# Autodesk Inventor assembly: Lotus_assembly
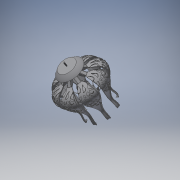
[picture p0: Inventor's stored thumbnail of the model, 180x180]
Saved by Autodesk Inventor 2019 (Build 230136000, 136)
## iProperties
Created: 2019-11-12
Part Number: Lotus_assembly
Document SubType Name: Assembly
Designer: Jorian Brusind
Author: Jorian Brusind
## Documents named in this file (9)
- C:\Users\Jorian Brusind\Documents\GitHub\PersonalProjects\Inventor Projects\Johan\Inventor Files\Lotus_assembly.iam
- C:\Users\Jorian Brusind\Documents\GitHub\PersonalProjects\Inventor Projects\Johan\Inventor Files\Lotus_Petal.ipt
- C:\Users\Jorian Brusind\Documents\GitHub\PersonalProjects\Inventor Projects\Johan\Inventor Files\Ring.ipt
- C:\Users\Jorian Brusind\Documents\GitHub\PersonalProjects\Inventor Projects\Johan\Inventor Files\Leaf.ipt
- C:\Users\Jorian Brusind\Documents\GitHub\PersonalProjects\Inventor Projects\Johan\Inventor Files\inner_ring.ipt
- C:\Users\Jorian Brusind\Documents\GitHub\PersonalProjects\Inventor Projects\Johan\Inventor Files\Innter_petal.ipt
- C:\Users\Jorian Brusind\Documents\GitHub\PersonalProjects\Inventor Projects\Johan\Inventor Files\Threaded_Rod.ipt
- C:\Users\Jorian Brusind\Documents\GitHub\PersonalProjects\Inventor Projects\Johan\Inventor Files\Hex_Center.ipt
- C:\Users\Jorian Brusind\Documents\GitHub\PersonalProjects\Inventor Projects\Johan\Inventor Files\Connector_Rd.ipt
## Components (25 placed, 8 different names)
1. Lotus_Petal:1 — Mate:6, Flush:8, Mate:29
2. Lotus_Petal:2 — Mate:2, Flush:6, Mate:33
3. Lotus_Petal:4 — Mate:4, Flush:1, Mate:27
4. Lotus_Petal:5 — Mate:1, Flush:4, Mate:37
5. Lotus_Petal:6 — Mate:3, Flush:5, Mate:35
6. Lotus_Petal:7 — Mate:5, Flush:7, Mate:31
7. Ring:1 — Mate:1, Mate:2, Mate:3, Mate:4, Mate:5, Mate:6, Mate:7, Mate:8, Flush:1, Flush:2, Flush:3, Flush:4, Flush:5, Flush:6, Flush:7, Flush:8, Mate:9, Mate:10, Mate:11, Mate:12, Mate:19
8. Lotus_Petal:8 — Mate:7, Flush:2, Mate:25
9. Lotus_Petal:9 — Mate:8, Flush:3, Mate:21, Mate:22
10. Leaf:1 — Mate:9, Mate:10, Flush:15
11. inner_ring:1 — Mate:11, Mate:12, Mate:13, Flush:9, Mate:14, Flush:10, Mate:15, Flush:11, Mate:16, Flush:12
12. Innter_petal:1 — Mate:13, Flush:9
13. Innter_petal:2 — Mate:16, Flush:12
14. Innter_petal:5 — Mate:14, Flush:10
15. Innter_petal:6 — Mate:15, Flush:11
16. Threaded_Rod:1 — Mate:19, Flush:15, Mate:20
17. Hex_Center:1 — Mate:20, Mate:23, Mate:24, Flush:16, Mate:26, Flush:17, Mate:28, Flush:18, Mate:30, Flush:19, Mate:32, Flush:20, Mate:34, Flush:21, Mate:36, Flush:22
18. Connector_Rd:1 — Mate:21, Mate:22, Mate:23
19. Connector_Rd:2 — Mate:36, Flush:22, Mate:37
20. Connector_Rd:3 — Mate:26, Flush:17, Mate:27
21. Connector_Rd:4 — Mate:24, Flush:16, Mate:25
22. Connector_Rd:5 — Mate:34, Flush:21, Mate:35
23. Connector_Rd:6 — Mate:32, Flush:20, Mate:33
24. Connector_Rd:7 — Mate:30, Flush:19, Mate:31
25. Connector_Rd:8 — Mate:28, Flush:18, Mate:29
## Relationships (55: Mate 35, Flush 20)
- Mate:1: Lotus_Petal:5 ↔ Ring:1
- Mate:2: Lotus_Petal:2 ↔ Ring:1
- Mate:3: Lotus_Petal:6 ↔ Ring:1
- Mate:4: Lotus_Petal:4 ↔ Ring:1
- Mate:5: Lotus_Petal:7 ↔ Ring:1
- Mate:6: Lotus_Petal:1 ↔ Ring:1
- Mate:7: Ring:1 ↔ Lotus_Petal:8
- Mate:8: Ring:1 ↔ Lotus_Petal:9
- Flush:1: Lotus_Petal:4 ↔ Ring:1
- Flush:2: Ring:1 ↔ Lotus_Petal:8
- Flush:3: Ring:1 ↔ Lotus_Petal:9
- Flush:4: Lotus_Petal:5 ↔ Ring:1
- Flush:5: Lotus_Petal:6 ↔ Ring:1
- Flush:6: Lotus_Petal:2 ↔ Ring:1
- Flush:7: Lotus_Petal:7 ↔ Ring:1
- Flush:8: Lotus_Petal:1 ↔ Ring:1
- Mate:9 (15 mm): Ring:1 ↔ Leaf:1
- Mate:10: Ring:1 ↔ Leaf:1
- Mate:11: Ring:1 ↔ inner_ring:1
- Mate:12 (30 mm): Ring:1 ↔ inner_ring:1
- Mate:13: inner_ring:1 ↔ Innter_petal:1
- Flush:9: inner_ring:1 ↔ Innter_petal:1
- Mate:14: inner_ring:1 ↔ Innter_petal:5
- Flush:10: inner_ring:1 ↔ Innter_petal:5
- Mate:15: inner_ring:1 ↔ Innter_petal:6
- Flush:11: inner_ring:1 ↔ Innter_petal:6
- Mate:16: inner_ring:1 ↔ Innter_petal:2
- Flush:12: inner_ring:1 ↔ Innter_petal:2
- Mate:19: Ring:1 ↔ Threaded_Rod:1
- Flush:15 (-10 mm): Leaf:1 ↔ Threaded_Rod:1
- Mate:20: Threaded_Rod:1 ↔ Hex_Center:1
- Mate:21: Lotus_Petal:9 ↔ Connector_Rd:1
- Mate:22 (0.25 mm): Lotus_Petal:9 ↔ Connector_Rd:1
- Mate:23: Hex_Center:1 ↔ Connector_Rd:1
- Mate:24: Hex_Center:1 ↔ Connector_Rd:4
- Flush:16 (-0.5 mm): Hex_Center:1 ↔ Connector_Rd:4
- Mate:25: Lotus_Petal:8 ↔ Connector_Rd:4
- Mate:26: Hex_Center:1 ↔ Connector_Rd:3
- Flush:17 (-0.5 mm): Hex_Center:1 ↔ Connector_Rd:3
- Mate:27: Lotus_Petal:4 ↔ Connector_Rd:3
- Mate:28: Hex_Center:1 ↔ Connector_Rd:8
- Flush:18 (-0.5 mm): Hex_Center:1 ↔ Connector_Rd:8
- Mate:29: Lotus_Petal:1 ↔ Connector_Rd:8
- Mate:30: Hex_Center:1 ↔ Connector_Rd:7
- Flush:19 (-0.5 mm): Hex_Center:1 ↔ Connector_Rd:7
- Mate:31: Lotus_Petal:7 ↔ Connector_Rd:7
- Mate:32: Hex_Center:1 ↔ Connector_Rd:6
- Flush:20 (-0.5 mm): Hex_Center:1 ↔ Connector_Rd:6
- Mate:33: Lotus_Petal:2 ↔ Connector_Rd:6
- Mate:34: Hex_Center:1 ↔ Connector_Rd:5
- Flush:21 (-0.5 mm): Hex_Center:1 ↔ Connector_Rd:5
- Mate:35: Lotus_Petal:6 ↔ Connector_Rd:5
- Mate:36: Hex_Center:1 ↔ Connector_Rd:2
- Flush:22 (-0.5 mm): Hex_Center:1 ↔ Connector_Rd:2
- Mate:37: Lotus_Petal:5 ↔ Connector_Rd:2
